# Autodesk Inventor assembly: Assembly_housing_V2
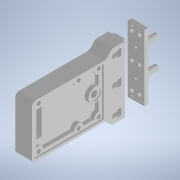
[picture p0: Inventor's stored thumbnail of the model, 180x180]
Saved by Autodesk Inventor 2020 (Build 240168000, 168)
## iProperties
Created: 2020-06-11
Part Number: Assembly_housing_V2
Document SubType Name: Assembly
Designer: Admin
Author: Admin
## Documents named in this file (3)
- C:\projets\wprop\WPropeller\Assembly_housing_V2.iam
- C:\PFE\interface_V2.ipt
- C:\PFE\housing_PCB_V3.ipt
## Components (2 placed, 2 different names)
1. interface_V2:1 — Mate:1, Mate:2, Mate:3
2. housing_PCB_V3:1 — Mate:1, Mate:2, Mate:3
## Relationships (3: Mate 3)
- Mate:1: interface_V2:1 ↔ housing_PCB_V3:1
- Mate:2: interface_V2:1 ↔ housing_PCB_V3:1
- Mate:3: interface_V2:1 ↔ housing_PCB_V3:1
